# Autodesk Inventor assembly: Shim_wearing_image
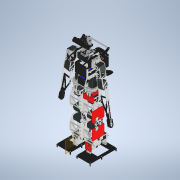
[picture p0: Inventor's stored thumbnail of the model, 180x180]
Saved by Autodesk Inventor 2020 (Build 240168000, 168)
## iProperties
Created: 2021-11-14
Part Number: Shim_wearing_image
Document SubType Name: Assembly
Designer: Masato Kubotera
Author: Masato Kubotera
## Documents named in this file (7)
- C:\Users\Masato\Documents\Inventor\CIT Brains_Inventor\OpenPlatform_ver3_0\Shim\Shim_wearing_image.iam
- C:\Users\Masato\Documents\Inventor\CIT Brains_Inventor\OpenPlatform_ver3_0\Body.iam
- C:\Users\Masato\Documents\Inventor\CIT Brains_Inventor\OpenPlatform_ver3_0\Shim\Knee_pitch_shim.ipt
- C:\Users\Masato\Documents\Inventor\CIT Brains_Inventor\OpenPlatform_ver3_0\Shim\Knee_pitch_shim_MIR.ipt
- C:\Users\Masato\Documents\Inventor\CIT Brains_Inventor\OpenPlatform_ver3_0\Shim\Leg_joint_roll.ipt
- C:\Users\Masato\Documents\Inventor\CIT Brains_Inventor\OpenPlatform_ver3_0\Shim\Leg_joint_yaw_shim.ipt
- C:\Users\Masato\Documents\Inventor\CIT Brains_Inventor\OpenPlatform_ver3_0\Shim\Ankle_roll_shim.ipt
## Components (6 placed, 6 different names)
1. Body:1 [sub-assembly] — 挿入:1, 角度:1, 挿入:2, 挿入:3, 角度:2, 角度:3, メイト:1, メイト:2, 角度:4, フラッシュ:4, フラッシュ:5, フラッシュ:6, 角度:5, メイト:3, メイト:4
2. Knee_pitch_shim:1 — 挿入:3, 角度:3
3. Knee_pitch_shim_MIR:1 — 挿入:2, 角度:2
4. Leg_joint_roll:1 — メイト:1, メイト:2, 角度:4
5. Leg_joint_yaw_shim:1 — 挿入:1, 角度:1
6. Ankle_roll_shim:1 — 角度:5, メイト:3, メイト:4
## Relationships (15: Angle 5, Mate 4, Insert 3, Flush 3)
- 挿入:1 [Insert]: Body:1 ↔ Leg_joint_yaw_shim:1
- 角度:1 [Angle] (0 deg): Body:1 ↔ Leg_joint_yaw_shim:1
- 挿入:2 [Insert]: Body:1 ↔ Knee_pitch_shim_MIR:1
- 挿入:3 [Insert]: Body:1 ↔ Knee_pitch_shim:1
- 角度:2 [Angle] (0 deg): Body:1 ↔ Knee_pitch_shim_MIR:1
- 角度:3 [Angle] (0 deg): Body:1 ↔ Knee_pitch_shim:1
- メイト:1 [Mate]: Body:1 ↔ Leg_joint_roll:1
- メイト:2 [Mate]: Body:1 ↔ Leg_joint_roll:1
- 角度:4 [Angle] (0 deg): Body:1 ↔ Leg_joint_roll:1
- フラッシュ:4 [Flush]: Body:1
- フラッシュ:5 [Flush]: Body:1
- フラッシュ:6 [Flush]: Body:1
- 角度:5 [Angle] (0 deg): Body:1 ↔ Ankle_roll_shim:1
- メイト:3 [Mate]: Body:1 ↔ Ankle_roll_shim:1
- メイト:4 [Mate]: Body:1 ↔ Ankle_roll_shim:1
